# Autodesk Inventor assembly: neo550
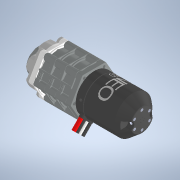
[picture p0: Inventor's stored thumbnail of the model, 180x180]
Saved by Autodesk Inventor 2020 (Build 240168000, 168)
## iProperties
Created: 2019-12-27
Part Number: neo550
Document SubType Name: Assembly
Designer: xj82b
Author: xj82b
## Documents named in this file (5)
- C:\Users\xj82b\Documents\Inventor\5199\neo550.iam
- C:\Users\xj82b\Documents\Inventor\5199\REV-21-1651.ipt
- C:\Users\xj82b\Documents\Inventor\5199\REV-41-1607.ipt
- C:\Users\xj82b\Documents\Inventor\5199\REV-41-1604.iam
- C:\Users\xj82b\Documents\Inventor\5199\REV-41-1603.iam
## Components (6 placed, 4 different names)
1. REV-21-1651:1 — Mate:1, Mate:2
2. REV-41-1607:1 — Mate:1, Mate:2, Mate:3, Flush:1, Flush:2
3. REV-41-1604:1 [sub-assembly] — Mate:10, Mate:11, Mate:12
4. REV-41-1603:1 [sub-assembly] — Mate:3, Flush:1, Flush:2, Mate:4, Mate:5, Mate:6
5. REV-41-1603:2 [sub-assembly] — Mate:4, Mate:5, Mate:6, Mate:7, Mate:8, Mate:9
6. REV-41-1603:3 [sub-assembly] — Mate:7, Mate:8, Mate:9, Mate:10, Mate:11, Mate:12
## Relationships (14: Mate 12, Flush 2)
- Mate:1: REV-21-1651:1 ↔ REV-41-1607:1
- Mate:2: REV-21-1651:1 ↔ REV-41-1607:1
- Mate:3: REV-41-1607:1 ↔ REV-41-1603:1
- Flush:1: REV-41-1607:1 ↔ REV-41-1603:1
- Flush:2: REV-41-1607:1 ↔ REV-41-1603:1
- Mate:4: REV-41-1603:1 ↔ REV-41-1603:2
- Mate:5: REV-41-1603:1 ↔ REV-41-1603:2
- Mate:6: REV-41-1603:1 ↔ REV-41-1603:2
- Mate:7: REV-41-1603:2 ↔ REV-41-1603:3
- Mate:8: REV-41-1603:2 ↔ REV-41-1603:3
- Mate:9: REV-41-1603:2 ↔ REV-41-1603:3
- Mate:10: REV-41-1604:1 ↔ REV-41-1603:3
- Mate:11: REV-41-1604:1 ↔ REV-41-1603:3
- Mate:12: REV-41-1604:1 ↔ REV-41-1603:3
